# Autodesk Inventor assembly: ASY MSC 080 gills
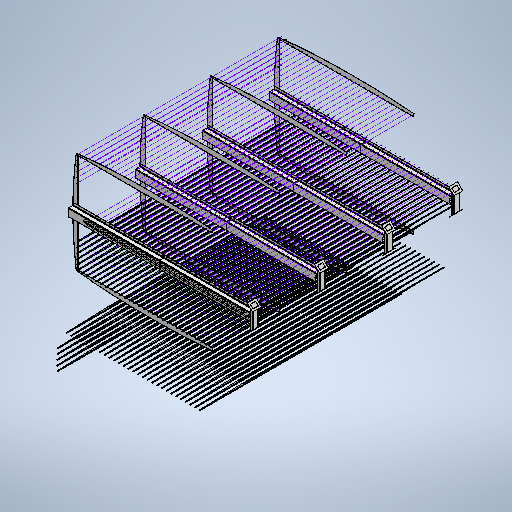
[picture p0: Inventor's stored thumbnail of the model, 512x512]
Saved by Autodesk Inventor 2025 (Build 290162010, 162A)
## iProperties
Created: 2024-08-31
Part Number: ASY MSC 080 gills
Document SubType Name: Assembly
Designer: pokla
Stock Number: ASY МОО 080 Жабры
Author: pokla
## Documents named in this file (20)
- C:\Users\user\YandexDisk\домашниий пк\Inventor\Manturovo\Manturovo_Se-clar\ASY MSC 080 gills.iam
- C:\Users\user\YandexDisk\домашниий пк\Inventor\Manturovo\Manturovo_Se-clar\MSC 802 sheet gills.ipt
- C:\Users\user\YandexDisk\домашниий пк\Inventor\Manturovo\Manturovo_Se-clar\MSC 081 pillar gills.ipt
- C:\Users\user\YandexDisk\домашниий пк\Inventor\Manturovo\Manturovo_Se-clar\MSC 804 sheet gills.ipt
- C:\Users\user\YandexDisk\домашниий пк\Inventor\Manturovo\Manturovo_Se-clar\MSC 803 sheet gills.ipt
- C:\Users\user\YandexDisk\домашниий пк\Inventor\Manturovo\Manturovo_Se-clar\MSC 806 sheet gills.ipt
- C:\Users\user\YandexDisk\домашниий пк\Inventor\Manturovo\Manturovo_Se-clar\MSC 805 sheet gills.ipt
- C:\Users\user\YandexDisk\домашниий пк\Inventor\Manturovo\Manturovo_Se-clar\MSC 808 sheet gills.ipt
- C:\Users\user\YandexDisk\домашниий пк\Inventor\Manturovo\Manturovo_Se-clar\MSC 807 sheet gills.ipt
- C:\Users\user\YandexDisk\домашниий пк\Inventor\Manturovo\Manturovo_Se-clar\MSC 810 sheet gills.ipt
- C:\Users\user\YandexDisk\домашниий пк\Inventor\Manturovo\Manturovo_Se-clar\MSC 809 sheet gills.ipt
- C:\Users\user\YandexDisk\домашниий пк\Inventor\Manturovo\Manturovo_Se-clar\MSC 812 sheet gills.ipt
- C:\Users\user\YandexDisk\домашниий пк\Inventor\Manturovo\Manturovo_Se-clar\MSC 811 sheet gills.ipt
- C:\Users\user\YandexDisk\домашниий пк\Inventor\Manturovo\Manturovo_Se-clar\MSC 084 wall support gills.ipt
- C:\Users\user\YandexDisk\домашниий пк\Inventor\Manturovo\Manturovo_Se-clar\MSC 082 pillar gills.ipt
- C:\Users\user\YandexDisk\домашниий пк\Inventor\Manturovo\Manturovo_Se-clar\MSC 086 string for sheets gills.ipt
- C:\Users\user\YandexDisk\домашниий пк\Inventor\Manturovo\Manturovo_Se-clar\MSC 083 top support gills.ipt
- C:\Users\user\YandexDisk\домашниий пк\Inventor\Manturovo\Manturovo_Se-clar\MSC 801 sheet gills.ipt
- C:\Users\user\YandexDisk\домашниий пк\Inventor\Manturovo\Manturovo_Se-clar\ASY MSC 089 gills base.iam
- C:\Users\user\YandexDisk\домашниий пк\Inventor\Manturovo\Manturovo_Se-clar\MSC 082 pillar 2.ipt
## Components (334 placed, 30 different names)
1. MSC 804 sheet gills:1 — Rigid:39
2. MSC 803 sheet gills:1 — Angle:2, Tangent:8, Tangent:9, Flush:15, Flush:19, Rigid:39
3. MSC 806 sheet gills:1 — Rigid:36
4. MSC 805 sheet gills:1 — Rigid:36, Angle:3, Tangent:10, Tangent:11, Flush:15, Flush:16
5. MSC 808 sheet gills:1 — Rigid:37
6. MSC 807 sheet gills:1 — Rigid:37, Angle:4, Tangent:12, Tangent:13, Flush:16, Flush:17
7. MSC 810 sheet gills:1 — Rigid:38
8. MSC 809 sheet gills:1 — Rigid:38, Angle:5, Tangent:17, Tangent:18, Flush:17, Flush:18
9. MSC 812 sheet gills:1 — Rigid:32
10. MSC 811 sheet gills:1 — Rigid:32, Angle:6, Tangent:19, Tangent:20, Flush:18
11. MSC 084 wall support gills:1 — Rigid:12, Rigid:25, Rigid:30, Tangent:14, Tangent:15
12. MSC 084 wall support gills:2 — Rigid:25, Rigid:26, Mate:17
13. MSC 084 wall support gills:3 — Rigid:26, Rigid:27
14. MSC 084 wall support gills:4 — Rigid:27
15. MSC 0103 sheet gills:2
16. MSC 0203 sheet gills:2
17. MSC 0104 sheet gills:2
18. MSC 0204 sheet gills:2
19. MSC 0105 sheet gills:2
20. MSC 0205 sheet gills:2
21. MSC 0106 sheet gills:2
22. MSC 0206 sheet gills:2
23. MSC 0107 sheet gills:2
24. MSC 0207 sheet gills:2
25. MSC 081 pillar gills:1 — Rotational:1, Rotational:2, Tangent:16, Mate:18
26. MSC 082 pillar gills:1 — Rigid:28, Rigid:29
27. ASY MSC 089 gills base:1 [sub-assembly]
28. MSC 083 top support gills:1 — Rigid:24, Rigid:29, Rigid:31
29. MSC 083 top support gills:2 — Rigid:28, Rigid:30, Tangent:8, Tangent:9, Tangent:10, Tangent:11, Tangent:12, Tangent:13, Tangent:17, Tangent:18, Tangent:19, Tangent:20, Rigid:40
30. MSC 084 wall support gills:5 — Rigid:15, Rigid:31
31. MSC 081 pillar gills:2
32. MSC 082 pillar gills:2
33. ASY MSC 089 gills base:2 [sub-assembly]
34. MSC 083 top support gills:3
35. MSC 083 top support gills:6
36. MSC 084 wall support gills:6
37. MSC 081 pillar gills:3
38. MSC 082 pillar gills:3
39. ASY MSC 089 gills base:3 [sub-assembly]
40. MSC 083 top support gills:4
41. MSC 083 top support gills:7
42. MSC 084 wall support gills:7
43. MSC 081 pillar gills:4
44. MSC 082 pillar gills:4
45. ASY MSC 089 gills base:4 [sub-assembly]
46. MSC 083 top support gills:5
47. MSC 083 top support gills:8
48. MSC 084 wall support gills:8
49. MSC 801 sheet gills:1 — Mate:17, Rigid:33, Angle:2, Angle:3, Angle:4, Angle:5, Angle:6, Tangent:14, Tangent:15, Tangent:16, Flush:19
50. MSC 802 sheet gills:1 — Rigid:33
51. MSC 802 sheet gills:2
52. MSC 0201 sheet gills:2
53. MSC 0201 sheet gills:3
54. MSC 802 sheet gills:3
55. MSC 802 sheet gills:4
56. MSC 0201 sheet gills:4
57. MSC 0201 sheet gills:5
58. MSC 802 sheet gills:5
59. MSC 802 sheet gills:6
60. MSC 0201 sheet gills:6
61. MSC 0201 sheet gills:7
62. MSC 802 sheet gills:7
63. MSC 802 sheet gills:8
64. MSC 0201 sheet gills:8
65. MSC 0201 sheet gills:9
66. MSC 802 sheet gills:9
67. MSC 802 sheet gills:10
68. MSC 0201 sheet gills:10
69. MSC 0201 sheet gills:11
70. MSC 802 sheet gills:11
71. MSC 802 sheet gills:12
72. MSC 0201 sheet gills:12
73. MSC 0201 sheet gills:13
74. MSC 802 sheet gills:13
75. MSC 802 sheet gills:14
76. MSC 0201 sheet gills:14
77. MSC 0201 sheet gills:15
78. MSC 802 sheet gills:15
79. MSC 802 sheet gills:16
80. MSC 0201 sheet gills:16
81. MSC 0201 sheet gills:17
82. MSC 802 sheet gills:17
83. MSC 802 sheet gills:18
84. MSC 0201 sheet gills:18
85. MSC 0201 sheet gills:19
86. MSC 802 sheet gills:19
87. MSC 802 sheet gills:20
88. MSC 0201 sheet gills:20
89. MSC 0201 sheet gills:21
90. MSC 802 sheet gills:21
91. MSC 802 sheet gills:22
92. MSC 0201 sheet gills:22
93. MSC 0201 sheet gills:23
94. MSC 802 sheet gills:23
95. MSC 802 sheet gills:24
96. MSC 0201 sheet gills:24
97. MSC 0201 sheet gills:25
98. MSC 802 sheet gills:25
99. MSC 802 sheet gills:26
100. MSC 0201 sheet gills:26
101. MSC 0201 sheet gills:27
102. MSC 802 sheet gills:27
103. MSC 802 sheet gills:28
104. MSC 0201 sheet gills:28
105. MSC 0201 sheet gills:29
106. MSC 802 sheet gills:29
107. MSC 802 sheet gills:30
108. MSC 0201 sheet gills:30
109. MSC 0201 sheet gills:31
110. MSC 802 sheet gills:31
111. MSC 802 sheet gills:32
112. MSC 0201 sheet gills:32
113. MSC 0201 sheet gills:33
114. MSC 802 sheet gills:33
115. MSC 802 sheet gills:34
116. MSC 0201 sheet gills:34
117. MSC 0201 sheet gills:35
118. MSC 802 sheet gills:35
119. MSC 802 sheet gills:36
120. MSC 0201 sheet gills:36
121. MSC 0201 sheet gills:37
122. MSC 802 sheet gills:37
123. MSC 802 sheet gills:38
124. MSC 0201 sheet gills:38
125. MSC 0201 sheet gills:39
126. MSC 802 sheet gills:39
127. MSC 802 sheet gills:40
128. MSC 0201 sheet gills:40
129. MSC 0201 sheet gills:41
130. MSC 802 sheet gills:41
131. MSC 802 sheet gills:42
132. MSC 0201 sheet gills:42
133. MSC 0201 sheet gills:43
134. MSC 802 sheet gills:43
135. MSC 802 sheet gills:44
136. MSC 0201 sheet gills:44
137. MSC 0201 sheet gills:45
138. MSC 802 sheet gills:45
139. MSC 802 sheet gills:46
140. MSC 0201 sheet gills:46
141. MSC 0201 sheet gills:47
142. MSC 802 sheet gills:47
143. MSC 802 sheet gills:48
144. MSC 0201 sheet gills:48
145. MSC 0201 sheet gills:49
146. MSC 802 sheet gills:49
147. MSC 802 sheet gills:50
148. MSC 0201 sheet gills:50
149. MSC 0201 sheet gills:51
150. MSC 802 sheet gills:51
151. MSC 802 sheet gills:52
152. MSC 0201 sheet gills:52
153. MSC 0201 sheet gills:53
154. MSC 802 sheet gills:53
155. MSC 802 sheet gills:54
156. MSC 0201 sheet gills:54
157. MSC 0201 sheet gills:55
158. MSC 802 sheet gills:55
159. MSC 802 sheet gills:56
160. MSC 0201 sheet gills:56
161. MSC 0201 sheet gills:57
162. MSC 802 sheet gills:57
163. MSC 802 sheet gills:58
164. MSC 0201 sheet gills:58
165. MSC 086 string for sheets gills:1 — Rigid:12
166. MSC 086 string for sheets gills:2 — Rigid:15
167. MSC 086 string for sheets gills:3
168. MSC 086 string for sheets gills:344
169. MSC 086 string for sheets gills:5
170. MSC 086 string for sheets gills:345
171. MSC 086 string for sheets gills:7
172. MSC 086 string for sheets gills:346
173. MSC 086 string for sheets gills:9
174. MSC 086 string for sheets gills:347
175. MSC 086 string for sheets gills:11
176. MSC 086 string for sheets gills:348
177. MSC 086 string for sheets gills:13
178. MSC 086 string for sheets gills:349
179. MSC 086 string for sheets gills:15
180. MSC 086 string for sheets gills:350
181. MSC 086 string for sheets gills:17
182. MSC 086 string for sheets gills:351
183. MSC 086 string for sheets gills:19
184. MSC 086 string for sheets gills:352
185. MSC 086 string for sheets gills:21
186. MSC 086 string for sheets gills:353
187. MSC 086 string for sheets gills:23
188. MSC 086 string for sheets gills:354
189. MSC 086 string for sheets gills:25
190. MSC 086 string for sheets gills:355
191. MSC 086 string for sheets gills:27
192. MSC 086 string for sheets gills:356
193. MSC 086 string for sheets gills:29
194. MSC 086 string for sheets gills:357
195. MSC 086 string for sheets gills:31
196. MSC 086 string for sheets gills:358
197. MSC 086 string for sheets gills:33
198. MSC 086 string for sheets gills:359
199. MSC 086 string for sheets gills:35
200. MSC 086 string for sheets gills:360
201. MSC 086 string for sheets gills:37
202. MSC 086 string for sheets gills:361
203. MSC 086 string for sheets gills:39
204. MSC 086 string for sheets gills:362
205. MSC 086 string for sheets gills:41
206. MSC 086 string for sheets gills:363
207. MSC 086 string for sheets gills:43
208. MSC 086 string for sheets gills:364
209. MSC 086 string for sheets gills:45
210. MSC 086 string for sheets gills:365
211. MSC 086 string for sheets gills:47
212. MSC 086 string for sheets gills:366
213. MSC 086 string for sheets gills:49
214. MSC 086 string for sheets gills:367
215. MSC 086 string for sheets gills:51
216. MSC 086 string for sheets gills:368
217. MSC 086 string for sheets gills:53
218. MSC 086 string for sheets gills:369
219. MSC 086 string for sheets gills:55
220. MSC 086 string for sheets gills:370
221. MSC 086 string for sheets gills:58 — Rotational:1
222. MSC 086 string for sheets gills:57 — Rotational:2
223. MSC 082 pillar 2:1 — Mate:18
224. MSC 086 string for sheets gills:278
225. MSC 086 string for sheets gills:279
226. MSC 082 pillar 2:2
227. MSC 086 string for sheets gills:280
228. MSC 086 string for sheets gills:281
229. MSC 082 pillar 2:3
230. MSC 086 string for sheets gills:282
231. MSC 086 string for sheets gills:283
232. MSC 082 pillar 2:4
233. MSC 086 string for sheets gills:284
234. MSC 086 string for sheets gills:285
235. MSC 082 pillar 2:5
236. MSC 086 string for sheets gills:286
237. MSC 086 string for sheets gills:287
238. MSC 082 pillar 2:6
239. MSC 086 string for sheets gills:288
240. MSC 086 string for sheets gills:289
241. MSC 082 pillar 2:7
242. MSC 086 string for sheets gills:290
243. MSC 086 string for sheets gills:291
244. MSC 082 pillar 2:8
245. MSC 086 string for sheets gills:292
246. MSC 086 string for sheets gills:293
247. MSC 082 pillar 2:9
248. MSC 086 string for sheets gills:294
249. MSC 086 string for sheets gills:295
250. MSC 082 pillar 2:10
251. MSC 086 string for sheets gills:296
252. MSC 086 string for sheets gills:297
253. MSC 082 pillar 2:11
254. MSC 086 string for sheets gills:298
255. MSC 086 string for sheets gills:299
256. MSC 082 pillar 2:12
257. MSC 086 string for sheets gills:300
258. MSC 086 string for sheets gills:301
259. MSC 082 pillar 2:13
260. MSC 086 string for sheets gills:302
261. MSC 086 string for sheets gills:303
262. MSC 082 pillar 2:14
263. MSC 086 string for sheets gills:304
264. MSC 086 string for sheets gills:305
265. MSC 082 pillar 2:15
266. MSC 086 string for sheets gills:306
267. MSC 086 string for sheets gills:307
268. MSC 082 pillar 2:16
269. MSC 086 string for sheets gills:308
270. MSC 086 string for sheets gills:309
271. MSC 082 pillar 2:17
272. MSC 086 string for sheets gills:310
273. MSC 086 string for sheets gills:311
274. MSC 082 pillar 2:18
275. MSC 086 string for sheets gills:312
276. MSC 086 string for sheets gills:313
277. MSC 082 pillar 2:19
278. MSC 086 string for sheets gills:314
279. MSC 086 string for sheets gills:315
280. MSC 082 pillar 2:20
281. MSC 086 string for sheets gills:316
282. MSC 086 string for sheets gills:317
283. MSC 082 pillar 2:21
284. MSC 086 string for sheets gills:318
285. MSC 086 string for sheets gills:319
286. MSC 082 pillar 2:22
287. MSC 086 string for sheets gills:320
288. MSC 086 string for sheets gills:321
289. MSC 082 pillar 2:23
290. MSC 086 string for sheets gills:322
291. MSC 086 string for sheets gills:323
292. MSC 082 pillar 2:24
293. MSC 086 string for sheets gills:324
294. MSC 086 string for sheets gills:325
295. MSC 082 pillar 2:25
296. MSC 086 string for sheets gills:326
297. MSC 086 string for sheets gills:327
298. MSC 082 pillar 2:26
299. MSC 086 string for sheets gills:328
300. MSC 086 string for sheets gills:329
301. MSC 082 pillar 2:27
302. MSC 086 string for sheets gills:330
303. MSC 086 string for sheets gills:331
304. MSC 082 pillar 2:28
305. MSC 086 string for sheets gills:332
306. MSC 086 string for sheets gills:333
307. MSC 082 pillar 2:29
308. MSC 086 string for sheets gills:334
309. MSC 086 string for sheets gills:335
310. MSC 082 pillar 2:30
311. MSC 086 string for sheets gills:336
312. MSC 086 string for sheets gills:337
313. MSC 082 pillar 2:31
314. MSC 086 string for sheets gills:338
315. MSC 086 string for sheets gills:339
316. MSC 082 pillar 2:32
317. MSC 086 string for sheets gills:340
318. MSC 086 string for sheets gills:341
319. MSC 082 pillar 2:33
320. MSC 086 string for sheets gills:342
321. MSC 086 string for sheets gills:343
322. MSC 082 pillar 2:34
323. MSC 086 string for sheets gills:125 — Rigid:40
324. MSC 086 string for sheets gills:126
325. MSC 086 string for sheets gills:127
326. MSC 086 string for sheets gills:128
327. MSC 086 string for sheets gills:129
328. MSC 086 string for sheets gills:130
329. MSC 086 string for sheets gills:131 — Rigid:24
330. MSC 086 string for sheets gills:371
331. MSC 086 string for sheets gills:372
332. MSC 086 string for sheets gills:373
333. MSC 086 string for sheets gills:374
334. MSC 086 string for sheets gills:375
## Component patterns: (4 elements, first: MSC 081 pillar gills:1 + MSC 082 pillar gills:1 + ASY MSC 089 gills base:1 + MSC 083 top support gills:1 + MSC 083 top support gills:2 + MSC 084 wall support gills:5), (29 elements, first: MSC 801 sheet gills:1 + MSC 802 sheet gills:1 + MSC 802 sheet gills:2 + MSC 0201 sheet gills:2), (28 elements, first: MSC 086 string for sheets gills:1 + MSC 086 string for sheets gills:2), (34 elements, first: MSC 086 string for sheets gills:58 + MSC 086 string for sheets gills:57 + MSC 082 pillar 2:1), (6 elements, first: MSC 086 string for sheets gills:125), (6 elements, first: MSC 086 string for sheets gills:131)
## Relationships (61: WeldJoint 24, Tangent 13, Flush 12, Mate 5, Angle 5, RevoluteJoint 2)
- [WeldJoint]: MSC 081 pillar gills:1 ↔ MSC 082 pillar gills:1
- [Flush]: MSC 081 pillar gills:1 ↔ ASY MSC 089 gills base:1
- [Mate]: MSC 081 pillar gills:1 ↔ ASY MSC 089 gills base:1
- [Flush] (5 mm): MSC 081 pillar gills:1 ↔ ASY MSC 089 gills base:1
- Rigid:12 [WeldJoint] (-5 mm): MSC 084 wall support gills:1 ↔ MSC 086 string for sheets gills:1
- Rigid:15 [WeldJoint] (-5 mm): MSC 084 wall support gills:5 ↔ MSC 086 string for sheets gills:2
- [Mate]: ASY MSC 089 gills base:1
- [Mate]: ASY MSC 089 gills base:1
- [Flush]: ASY MSC 089 gills base:1
- Rigid:24 [WeldJoint] (-5 mm): MSC 083 top support gills:1 ↔ MSC 086 string for sheets gills:131
- Rigid:25 [WeldJoint] (985 mm): MSC 084 wall support gills:1 ↔ MSC 084 wall support gills:2
- Rigid:26 [WeldJoint] (985 mm): MSC 084 wall support gills:2 ↔ MSC 084 wall support gills:3
- Rigid:27 [WeldJoint] (985 mm): MSC 084 wall support gills:3 ↔ MSC 084 wall support gills:4
- Mate:17: MSC 084 wall support gills:2 ↔ MSC 801 sheet gills:1
- Rigid:28 [WeldJoint]: MSC 082 pillar gills:1 ↔ MSC 083 top support gills:2
- Rigid:29 [WeldJoint]: MSC 082 pillar gills:1 ↔ MSC 083 top support gills:1
- Rigid:30 [WeldJoint]: MSC 084 wall support gills:1 ↔ MSC 083 top support gills:2
- Rigid:31 [WeldJoint]: MSC 083 top support gills:1 ↔ MSC 084 wall support gills:5
- Rotational:1 [RevoluteJoint] (5 mm): MSC 081 pillar gills:1 ↔ MSC 086 string for sheets gills:58
- Rotational:2 [RevoluteJoint] (-5 mm): MSC 081 pillar gills:1 ↔ MSC 086 string for sheets gills:57
- Rigid:32 [WeldJoint] (-10 mm): MSC 812 sheet gills:1 ↔ MSC 811 sheet gills:1
- Rigid:33 [WeldJoint] (-10 mm): MSC 801 sheet gills:1 ↔ MSC 802 sheet gills:1
- Rigid:36 [WeldJoint] (-10 mm): MSC 806 sheet gills:1 ↔ MSC 805 sheet gills:1
- Rigid:37 [WeldJoint] (-10 mm): MSC 808 sheet gills:1 ↔ MSC 807 sheet gills:1
- Rigid:38 [WeldJoint] (-10 mm): MSC 810 sheet gills:1 ↔ MSC 809 sheet gills:1
- Angle:2 (0 deg): MSC 803 sheet gills:1 ↔ MSC 801 sheet gills:1
- Angle:3 (0 deg): MSC 805 sheet gills:1 ↔ MSC 801 sheet gills:1
- Angle:4 (0 deg): MSC 807 sheet gills:1 ↔ MSC 801 sheet gills:1
- Angle:5 (0 deg): MSC 809 sheet gills:1 ↔ MSC 801 sheet gills:1
- Angle:6 (0 deg): MSC 811 sheet gills:1 ↔ MSC 801 sheet gills:1
- Tangent:8: MSC 803 sheet gills:1 ↔ MSC 083 top support gills:2
- Tangent:9: MSC 803 sheet gills:1 ↔ MSC 083 top support gills:2
- Tangent:10: MSC 805 sheet gills:1 ↔ MSC 083 top support gills:2
- Tangent:11: MSC 805 sheet gills:1 ↔ MSC 083 top support gills:2
- Tangent:12: MSC 807 sheet gills:1 ↔ MSC 083 top support gills:2
- Tangent:13: MSC 807 sheet gills:1 ↔ MSC 083 top support gills:2
- Tangent:14: MSC 084 wall support gills:1 ↔ MSC 801 sheet gills:1
- Tangent:15: MSC 084 wall support gills:1 ↔ MSC 801 sheet gills:1
- Tangent:16: MSC 081 pillar gills:1 ↔ MSC 801 sheet gills:1
- Tangent:17: MSC 809 sheet gills:1 ↔ MSC 083 top support gills:2
- Tangent:18: MSC 809 sheet gills:1 ↔ MSC 083 top support gills:2
- Tangent:19: MSC 811 sheet gills:1 ↔ MSC 083 top support gills:2
- Tangent:20: MSC 811 sheet gills:1 ↔ MSC 083 top support gills:2
- Flush:15: MSC 803 sheet gills:1 ↔ MSC 805 sheet gills:1
- Flush:16: MSC 805 sheet gills:1 ↔ MSC 807 sheet gills:1
- Flush:17: MSC 807 sheet gills:1 ↔ MSC 809 sheet gills:1
- Flush:18: MSC 809 sheet gills:1 ↔ MSC 811 sheet gills:1
- Flush:19: MSC 803 sheet gills:1 ↔ MSC 801 sheet gills:1
- Rigid:39 [WeldJoint] (-10 mm): MSC 804 sheet gills:1 ↔ MSC 803 sheet gills:1
- Rigid:40 [WeldJoint] (5 mm): MSC 083 top support gills:2 ↔ MSC 086 string for sheets gills:125
- [WeldJoint] (-10 mm): MSC 802 sheet gills:2 ↔ MSC 0201 sheet gills:2
- [WeldJoint] (-10 mm): MSC 0107 sheet gills:2 ↔ MSC 0207 sheet gills:2
- [WeldJoint] (-10 mm): MSC 0104 sheet gills:2 ↔ MSC 0204 sheet gills:2
- [WeldJoint] (-10 mm): MSC 0105 sheet gills:2 ↔ MSC 0205 sheet gills:2
- [WeldJoint] (-10 mm): MSC 0106 sheet gills:2 ↔ MSC 0206 sheet gills:2
- [Flush]: MSC 0203 sheet gills:2 ↔ MSC 0204 sheet gills:2
- [Flush]: MSC 0204 sheet gills:2 ↔ MSC 0205 sheet gills:2
- [Flush]: MSC 0205 sheet gills:2 ↔ MSC 0206 sheet gills:2
- [Flush]: MSC 0206 sheet gills:2 ↔ MSC 0207 sheet gills:2
- [WeldJoint] (-10 mm): MSC 0103 sheet gills:2 ↔ MSC 0203 sheet gills:2
- Mate:18: MSC 081 pillar gills:1 ↔ MSC 082 pillar 2:1
## Named parameters: d233_d176 = -10 mm, d234_d202 = 0 mm, d235_d203 = 0 mm, d236_d204 = 0 mm, d237_d205 = 0 mm, d238_d207 = -10 mm, d239_d180 = -10 mm, d240_d181 = -10 mm, d241_d173 = -10 mm, d242_d179 = -10 mm
